# Autodesk Inventor assembly: TestAssembly1
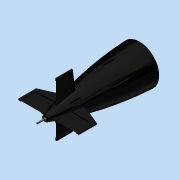
[picture p0: Inventor's stored thumbnail of the model, 180x180]
Saved by Autodesk Inventor 2017 (Build 210142000, 142)
## iProperties
Created: 2016-10-16
Part Number: TestAssembly1
Document SubType Name: Assembly
Designer: techn
Author: techn
## Documents named in this file (5)
- D:\OneDrive\Documents\Other Projects\Submarine\CAD\aft\TestAssembly1.iam
- D:\OneDrive\Documents\Other Projects\Submarine\CAD\aft\AftSectionAirtightRear.ipt
- D:\OneDrive\Documents\Other Projects\Submarine\CAD\aft\AftSectionWithSteeringLinkages.ipt
- D:\OneDrive\Documents\Other Projects\Submarine\CAD\aft\MotorAssembly0.iam
- D:\OneDrive\Documents\Other Projects\Submarine\CAD\aft\RearmostAftSectionAssembly0.iam
## Components (4 placed, 4 different names)
1. AftSectionAirtightRear:1 — Mate:1, Mate:2, Mate:5, Mate:6
2. AftSectionWithSteeringLinkages:1 — Mate:1, Mate:2, Mate:3, Mate:4
3. MotorAssembly0:1 [sub-assembly] — Mate:5, Mate:6
4. RearmostAftSectionAssembly0:1 [sub-assembly] — Mate:3, Mate:4
## Relationships (6: Mate 6)
- Mate:1: AftSectionAirtightRear:1 ↔ AftSectionWithSteeringLinkages:1
- Mate:2: AftSectionAirtightRear:1 ↔ AftSectionWithSteeringLinkages:1
- Mate:3: AftSectionWithSteeringLinkages:1 ↔ RearmostAftSectionAssembly0:1
- Mate:4: AftSectionWithSteeringLinkages:1 ↔ RearmostAftSectionAssembly0:1
- Mate:5: AftSectionAirtightRear:1 ↔ MotorAssembly0:1
- Mate:6: AftSectionAirtightRear:1 ↔ MotorAssembly0:1
